# Autodesk Inventor assembly: Lathe Model V3
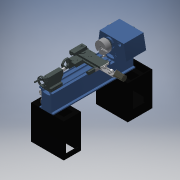
[picture p0: Inventor's stored thumbnail of the model, 180x180]
Saved by Autodesk Inventor 2016 (Build 200138000, 138)
## iProperties
Created: 2017-05-02
Part Number: Lathe Model V3
Document SubType Name: Assembly
Designer: M228544
Author: M228544
## Documents named in this file (26)
- C:\Users\M227562\Documents\GitHub\CNC-Lathe-CAD\Lathe with updated parts (LATEST of 20 06 17)\Lathe Model V3.iam
- C:\Users\M227562\Documents\GitHub\CNC-Lathe-CAD\Lathe with updated parts (LATEST of 20 06 17)\BED.ipt
- C:\Users\M227562\Documents\GitHub\CNC-Lathe-CAD\Lathe with updated parts (LATEST of 20 06 17)\saddle.ipt
- C:\Users\M227562\Documents\GitHub\CNC-Lathe-CAD\Lathe with updated parts (LATEST of 20 06 17)\Bottom-Tool-Bit.ipt
- C:\Users\M227562\Documents\GitHub\CNC-Lathe-CAD\Lathe with updated parts (LATEST of 20 06 17)\Top-Part-Tool-bit.ipt
- C:\Users\M227562\Documents\GitHub\CNC-Lathe-CAD\Lathe with updated parts (LATEST of 20 06 17)\slide-ontop-of-saddle.ipt
- C:\Users\M227562\Documents\GitHub\CNC-Lathe-CAD\Lathe with updated parts (LATEST of 20 06 17)\tail stock - body part.ipt
- C:\Users\M227562\Documents\GitHub\CNC-Lathe-CAD\Lathe with updated parts (LATEST of 20 06 17)\Gearbox.ipt
- C:\Users\M227562\Documents\GitHub\CNC-Lathe-CAD\Lathe with updated parts (LATEST of 20 06 17)\Left leg.ipt
- C:\Users\M227562\Documents\GitHub\CNC-Lathe-CAD\Lathe with updated parts (LATEST of 20 06 17)\Right Leg.ipt
- C:\Users\M227562\Documents\GitHub\CNC-Lathe-CAD\Lathe with updated parts (LATEST of 20 06 17)\Apron.ipt
- C:\Users\M227562\Documents\GitHub\CNC-Lathe-CAD\Lathe with updated parts (LATEST of 20 06 17)\AIS2016\BNT 2010-2_6 +1166L C7T-J1K_10000KBK 15BF 15.iam
- C:\Users\M227562\Documents\GitHub\CNC-Lathe-CAD\Lathe with updated parts (LATEST of 20 06 17)\Servo Motor\Servo Motor.iam
- C:\Users\M227562\Documents\GitHub\CNC-Lathe-CAD\Lathe with updated parts (LATEST of 20 06 17)\Support main frame motor-ball screw.ipt
- C:\Users\M227562\Documents\GitHub\CNC-Lathe-CAD\Lathe with updated parts (LATEST of 20 06 17)\Internal support motor-ball bracket.ipt
- C:\Users\M227562\Documents\GitHub\CNC-Lathe-CAD\Lathe with updated parts (LATEST of 20 06 17)\Motor support.ipt
- C:\Users\M227562\Documents\GitHub\CNC-Lathe-CAD\Lathe with updated parts (LATEST of 20 06 17)\Ball screw right hand support.ipt
- C:\Users\M227562\Documents\GitHub\CNC-Lathe-CAD\Lathe with updated parts (LATEST of 20 06 17)\Ball screw nut and apron join.ipt
- C:\Users\M227562\Documents\GitHub\CNC-Lathe-CAD\Lathe with updated parts (LATEST of 20 06 17)\barrel.ipt
- C:\Users\M227562\Documents\GitHub\CNC-Lathe-CAD\Lathe with updated parts (LATEST of 20 06 17)\connecting wheel.ipt
- C:\Users\M227562\Documents\GitHub\CNC-Lathe-CAD\Lathe with updated parts (LATEST of 20 06 17)\chuck holder.ipt
- C:\Users\M227562\Documents\GitHub\CNC-Lathe-CAD\Lathe with updated parts (LATEST of 20 06 17)\Chuck shaft.ipt
- C:\Users\M227562\Documents\GitHub\CNC-Lathe-CAD\Lathe with updated parts (LATEST of 20 06 17)\short shaft x axis\shaft and nut.iam
- C:\Users\M227562\Documents\GitHub\CNC-Lathe-CAD\Lathe with updated parts (LATEST of 20 06 17)\X axis screw support.ipt
- C:\Users\M227562\Documents\GitHub\CNC-Lathe-CAD\Chucks\3 jaw\Assembly3.iam
- C:\Users\M227562\Documents\GitHub\CNC-Lathe-CAD\Gearbox Handle and other bits\Gearbox Handle.iam
## Components (26 placed, 25 different names)
1. BED:1 — Mate:1, Mate:2, Mate:9, Mate:10, Mate:11, Flush:5, Flush:6, Mate:13, Mate:14, Flush:7, Flush:9, Mate:22, Mate:23, Flush:15, Flush:28, Flush:29, Mate:30, Mate:31, Mate:32, Mate:33
2. saddle:1 — Mate:1, Mate:2, Mate:5, Mate:6, Saddle and Slice on top of saddle, Flush:10, Flush:11, Mate:15, Mate:20, Angle:5, Mate:44, Angle:6, Flush:36, Angle:7
3. Bottom-Tool-Bit:1 — Mate:3, Mate:4, Flush:14
4. Top-Part-Tool-bit:1 — Mate:3, Mate:4, Mate:7, Mate:8, Tool Bit and Slece on top of saddle, Flush:14
5. slide-ontop-of-saddle:1 — Mate:5, Mate:6, Mate:7, Mate:8, Saddle and Slice on top of saddle, Tool Bit and Slece on top of saddle, Flush:34, Flush:35, Mate:43
6. tail stock - body part:1 — Mate:9, Mate:10, Flush:13, Mate:19, Mate:20, Mate:35, Mate:38, Flush:33
7. Gearbox:1 — Mate:11, Flush:5, Flush:13, Mate:19, Mate:21, Mate:39, Mate:40, Rotational:1
8. Left leg:1 — Mate:14, Flush:7, Flush:8
9. Right Leg:1 — Flush:6, Mate:13, Flush:8, Flush:9
10. Apron:1 — Flush:10, Flush:11, Mate:15, Mate:21, Flush:16, Angle:2, Mate:34
11. BNT 2010-2_6 +1166L C7T-J1K_10000KBK 15BF 15:1 [sub-assembly] — Mate:22, Mate:23, Flush:15, Mate:24, Mate:25, Flush:16, Angle:2, Mate:26, Flush:31, Flush:32
12. Servo Motor:1 [sub-assembly] — Mate:24, Mate:25, Mate:28, Angle:3, Mate:29
13. Support Motor-ball screw main frame — Flush:28, Flush:29, Flush:30, Mate:27, Angle:4, Mate:30
14. Internal support motor-ball bracket:1 — Mate:26, Flush:30, Mate:27
15. Motor support:1 — Mate:28, Angle:3, Mate:29, Angle:4
16. Ball screw right hand support:1 — Mate:31, Mate:32, Mate:33
17. Ball screw nut and apron join:1 — Mate:34, Flush:31, Flush:32
18. barrel:1 — Mate:35, Mate:36, Mate:37, Rotation/Translation:1, Flush:33
19. connecting wheel:1 — Mate:36, Mate:37, Mate:38, Rotation/Translation:1
20. chuck holder:1 — Mate:39, Mate:40, Mate:41, Mate:42, Mate:48
21. Chuck shaft:1 — Mate:41, Mate:42, Mate:47
22. shaft and nut:1 [sub-assembly] — Flush:34, Flush:35, Mate:43, Angle:5, Mate:44, Angle:6, Mate:45
23. X axis screw support:1 — Flush:36, Mate:46
24. Servo Motor:2 [sub-assembly] — Mate:45, Mate:46, Angle:7
25. Assembly3:1 [sub-assembly] — Mate:47, Mate:48
26. Gearbox Handle:1 [sub-assembly] — Rotational:1
## Relationships (74: Mate 44, Flush 21, Angle 7, RelateRotateTranslate 1, RevoluteJoint 1)
- Mate:1: BED:1 ↔ saddle:1
- Mate:2: BED:1 ↔ saddle:1
- Mate:3: Bottom-Tool-Bit:1 ↔ Top-Part-Tool-bit:1
- Mate:4: Bottom-Tool-Bit:1 ↔ Top-Part-Tool-bit:1
- Mate:5: saddle:1 ↔ slide-ontop-of-saddle:1
- Mate:6: saddle:1 ↔ slide-ontop-of-saddle:1
- Mate:7: Top-Part-Tool-bit:1 ↔ slide-ontop-of-saddle:1
- Mate:8: Top-Part-Tool-bit:1 ↔ slide-ontop-of-saddle:1
- Mate:9: BED:1 ↔ tail stock - body part:1
- Mate:10: BED:1 ↔ tail stock - body part:1
- Saddle and Slice on top of saddle [Flush]: saddle:1 ↔ slide-ontop-of-saddle:1
- Tool Bit and Slece on top of saddle [Angle] (-90 deg): Top-Part-Tool-bit:1 ↔ slide-ontop-of-saddle:1
- Mate:11: BED:1 ↔ Gearbox:1
- Flush:5: BED:1 ↔ Gearbox:1
- Flush:13: tail stock - body part:1 ↔ Gearbox:1
- Flush:6: BED:1 ↔ Right Leg:1
- Mate:13: BED:1 ↔ Right Leg:1
- Mate:14: BED:1 ↔ Left leg:1
- Flush:7: BED:1 ↔ Left leg:1
- Flush:8: Left leg:1 ↔ Right Leg:1
- Flush:9 (145 mm): BED:1 ↔ Right Leg:1
- Flush:10: saddle:1 ↔ Apron:1
- Flush:11: saddle:1 ↔ Apron:1
- Mate:15: saddle:1 ↔ Apron:1
- Flush:14: Bottom-Tool-Bit:1 ↔ Top-Part-Tool-bit:1
- Mate:19: tail stock - body part:1 ↔ Gearbox:1
- Mate:20: saddle:1 ↔ tail stock - body part:1
- Mate:21: Gearbox:1 ↔ Apron:1
- Mate:22 (-3 mm): BED:1 ↔ BNT 2010-2_6 +1166L C7T-J1K_10000KBK 15BF 15:1
- Mate:23 (15 mm): BED:1 ↔ BNT 2010-2_6 +1166L C7T-J1K_10000KBK 15BF 15:1
- Flush:15 (10 mm): BED:1 ↔ BNT 2010-2_6 +1166L C7T-J1K_10000KBK 15BF 15:1
- Mate:24: BNT 2010-2_6 +1166L C7T-J1K_10000KBK 15BF 15:1 ↔ Servo Motor:1
- Mate:25 (1 mm): BNT 2010-2_6 +1166L C7T-J1K_10000KBK 15BF 15:1 ↔ Servo Motor:1
- Flush:16 (5 mm): Apron:1 ↔ BNT 2010-2_6 +1166L C7T-J1K_10000KBK 15BF 15:1
- Angle:2 (180 deg): Apron:1 ↔ BNT 2010-2_6 +1166L C7T-J1K_10000KBK 15BF 15:1
- Mate:26: BNT 2010-2_6 +1166L C7T-J1K_10000KBK 15BF 15:1 ↔ Internal support motor-ball bracket:1
- Flush:28: BED:1 ↔ Support Motor-ball screw main frame
- Flush:29: BED:1 ↔ Support Motor-ball screw main frame
- Flush:30 (3 mm): Support Motor-ball screw main frame ↔ Internal support motor-ball bracket:1
- Mate:27 (-7 mm): Support Motor-ball screw main frame ↔ Internal support motor-ball bracket:1
- Mate:28: Servo Motor:1 ↔ Motor support:1
- Angle:3 (0 deg): Servo Motor:1 ↔ Motor support:1
- Mate:29: Servo Motor:1 ↔ Motor support:1
- Angle:4 (180 deg): Support Motor-ball screw main frame ↔ Motor support:1
- Mate:30: BED:1 ↔ Support Motor-ball screw main frame
- Mate:31: BED:1 ↔ Ball screw right hand support:1
- Mate:32: BED:1 ↔ Ball screw right hand support:1
- Mate:33: BED:1 ↔ Ball screw right hand support:1
- Mate:34: Apron:1 ↔ Ball screw nut and apron join:1
- Flush:31: BNT 2010-2_6 +1166L C7T-J1K_10000KBK 15BF 15:1 ↔ Ball screw nut and apron join:1
- Flush:32: BNT 2010-2_6 +1166L C7T-J1K_10000KBK 15BF 15:1 ↔ Ball screw nut and apron join:1
- Mate:35: tail stock - body part:1 ↔ barrel:1
- Mate:36: barrel:1 ↔ connecting wheel:1
- Mate:37: barrel:1 ↔ connecting wheel:1
- Mate:38: tail stock - body part:1 ↔ connecting wheel:1
- Rotation/Translation:1 [RelateRotateTranslate] (100 mm): barrel:1 ↔ connecting wheel:1
- Flush:33: tail stock - body part:1 ↔ barrel:1
- Mate:39: Gearbox:1 ↔ chuck holder:1
- Mate:40 (0.46 mm): Gearbox:1 ↔ chuck holder:1
- Mate:41: chuck holder:1 ↔ Chuck shaft:1
- Mate:42 (11.2 mm): chuck holder:1 ↔ Chuck shaft:1
- Flush:34: slide-ontop-of-saddle:1 ↔ shaft and nut:1
- Flush:35: slide-ontop-of-saddle:1 ↔ shaft and nut:1
- Mate:43: slide-ontop-of-saddle:1 ↔ shaft and nut:1
- Angle:5 (0 deg): saddle:1 ↔ shaft and nut:1
- Mate:44: saddle:1 ↔ shaft and nut:1
- Angle:6 (0 deg): saddle:1 ↔ shaft and nut:1
- Flush:36: saddle:1 ↔ X axis screw support:1
- Mate:45: shaft and nut:1 ↔ Servo Motor:2
- Mate:46: X axis screw support:1 ↔ Servo Motor:2
- Angle:7 (225 deg): saddle:1 ↔ Servo Motor:2
- Mate:47: Chuck shaft:1 ↔ Assembly3:1
- Mate:48: chuck holder:1 ↔ Assembly3:1
- Rotational:1 [RevoluteJoint]: Gearbox:1 ↔ Gearbox Handle:1
